# Autodesk Inventor assembly: TAZ 6 Assembly
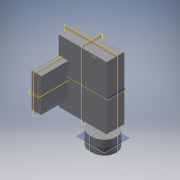
[picture p0: Inventor's stored thumbnail of the model, 180x180]
Saved by Autodesk Inventor 2019 (Build 230136000, 136)
## iProperties
Created: 2021-05-09
Part Number: TAZ 6 Assembly
Document SubType Name: Assembly
Designer: Eric
Author: Eric
## Documents named in this file (4)
- C:\Users\Eric\Documents\! - Uni\Year 4\MENG-Robot-Fab-Project\Models\For_Optimiser\Static Parts Assembly\TAZ 6 Assembly\TAZ 6 Assembly.iam
- C:\Users\Eric\Documents\! - Uni\Year 4\MENG-Robot-Fab-Project\Models\For_Optimiser\Static Parts Assembly\TAZ 6 Assembly\TAZ 6 Spool Convex Model.ipt
- C:\Users\Eric\Documents\! - Uni\Year 4\MENG-Robot-Fab-Project\Models\For_Optimiser\Static Parts Assembly\TAZ 6 Assembly\TAZ 6 Gantry Convex Model.iam
- C:\Users\Eric\Documents\! - Uni\Year 4\MENG-Robot-Fab-Project\Models\For_Optimiser\Static Parts Assembly\TAZ 6 Assembly\TAZ 6 Plate Convex Model.iam
## Components (3 placed, 3 different names)
1. TAZ 6 Gantry Convex Model:2 [sub-assembly] — Flush:3, Flush:7, Mate:6, Mate:7, Mate:8, Mate:9
2. TAZ 6 Plate Convex Model:2 [sub-assembly] — Flush:3, Flush:7, Mate:6
3. TAZ 6 Spool Convex Model:2 — Mate:7, Mate:8, Mate:9
## Relationships (6: Mate 4, Flush 2)
- Flush:3: TAZ 6 Gantry Convex Model:2 ↔ TAZ 6 Plate Convex Model:2
- Flush:7 (42.19 mm): TAZ 6 Gantry Convex Model:2 ↔ TAZ 6 Plate Convex Model:2
- Mate:6 (37.598 mm): TAZ 6 Gantry Convex Model:2 ↔ TAZ 6 Plate Convex Model:2
- Mate:7 (61.41 mm): TAZ 6 Gantry Convex Model:2 ↔ TAZ 6 Spool Convex Model:2
- Mate:8 (186 mm): TAZ 6 Gantry Convex Model:2 ↔ TAZ 6 Spool Convex Model:2
- Mate:9: TAZ 6 Gantry Convex Model:2 ↔ TAZ 6 Spool Convex Model:2
